# Autodesk Inventor assembly: Base Cover Assembly
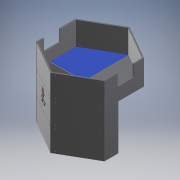
[picture p0: Inventor's stored thumbnail of the model, 180x180]
Saved by Autodesk Inventor 2017 (Build 210142000, 142)
## iProperties
Created: 2018-10-18
Part Number: Base Cover Assembly
Document SubType Name: Assembly
Designer: Dell
Author: Dell
## Documents named in this file (15)
- C:\Users\Dell\Documents\GitHub\tr2\Base\Base Cover Assembly.iam
- C:\Users\Dell\Documents\GitHub\tr2\Base\BA03.ipt
- C:\Users\Dell\Documents\GitHub\tr2\Base\BA04.ipt
- C:\Users\Dell\Documents\GitHub\tr2\Base\BA05.ipt
- C:\Users\Dell\Documents\GitHub\tr2\Base\BA09.ipt
- C:\Users\Dell\Documents\GitHub\tr2\Base\BA10.ipt
- C:\Users\Dell\Documents\GitHub\tr2\Base\BA12.ipt
- C:\Users\Dell\Documents\GitHub\tr2\Base\BA14.ipt
- C:\Users\Dell\Documents\GitHub\tr2\Base\Power Switch\Power Switch.iam
- C:\Users\Dell\Documents\GitHub\tr2\Base\Ethernet Port.ipt
- C:\Users\Dell\Documents\GitHub\tr2\Base\HDMI Port.ipt
- C:\Users\Dell\Documents\GitHub\tr2\Base\USB Hub.ipt
- C:\Users\Dell\Documents\GitHub\tr2\Base\BA19.ipt
- C:\Users\Dell\Documents\GitHub\tr2\Base\BA20.ipt
- C:\Users\Dell\Documents\GitHub\tr2\Base\BA21.ipt
## Components (24 placed, 14 different names)
1. BA03:1 — Mate:38, Mate:41, Flush:10, Mate:52, Mate:55
2. BA03:2 — Mate:20, Mate:43, Mate:44, Flush:10
3. BA03:3 — Mate:21, Mate:22, Mate:26, Mate:53
4. BA03:4 — Mate:17, Mate:19, Mate:21, Mate:23, Mate:64, Mate:65
5. BA04:1 — Mate:24, Mate:25, Mate:26, Mate:29, Mate:30
6. BA05:1 — Mate:18, Mate:19, Mate:20, Mate:23, Mate:27, Mate:66
7. BA03:5 — Mate:36, Mate:38, Mate:47
8. BA03:6 — Mate:41, Mate:49, Mate:81, Mate:83
9. BA03:7 — Mate:43, Mate:44, Mate:56, Mate:80
10. BA09:1 — Mate:29, Mate:30, Mate:33
11. BA09:4 — Mate:27, Mate:34, Mate:36
12. BA10:1 — Mate:17, Mate:18, Mate:22, Mate:24, Mate:25
13. BA10:2 — Mate:64, Mate:65, Mate:66
14. BA12:1 — Mate:33, Mate:54, Mate:75
15. BA12:2 — Mate:34, Mate:76
16. BA14:1 — Mate:47, Mate:49, Mate:55, Mate:56, Mate:57, Mate:58, Mate:59, Mate:67, Mate:68, Flush:11, Mate:69, Mate:70, Mate:71, Mate:72, Flush:12, Flush:13
17. Power Switch:1 [sub-assembly] — Mate:57, Mate:58, Mate:59
18. Ethernet Port:1 — Mate:69, Mate:72, Flush:13
19. HDMI Port:1 — Mate:70, Mate:71, Flush:12
20. USB Hub:1 — Mate:67, Mate:68, Flush:11
21. BA19:1 — Mate:75, Mate:78, Mate:85
22. BA19:2 — Mate:76, Mate:85
23. BA20:1 — Mate:78, Mate:80
24. BA21:1 — Mate:81, Mate:83
## Relationships (59: Mate 53, Flush 6)
- [Mate]: BA03:3 ↔ BA03:4
- [Mate]: BA03:2 ↔ BA03:5
- [Mate]: BA03:5 ↔ BA03:6
- [Mate]: BA04:1 ↔ BA09:1
- [Mate]: BA05:1 ↔ BA09:4
- [Mate]: BA04:1 ↔ BA12:1
- [Mate]: BA05:1 ↔ BA12:2
- [Flush]: BA09:4 ↔ BA12:2
- [Flush]: BA03:3 ↔ BA10:1
- Mate:17: BA03:4 ↔ BA10:1
- Mate:18: BA05:1 ↔ BA10:1
- Mate:19: BA03:4 ↔ BA05:1
- Mate:20: BA03:2 ↔ BA05:1
- Mate:21: BA03:3 ↔ BA03:4
- Mate:22: BA03:3 ↔ BA10:1
- Mate:23: BA03:4 ↔ BA05:1
- Mate:24: BA04:1 ↔ BA10:1
- Mate:25: BA04:1 ↔ BA10:1
- Mate:26: BA03:3 ↔ BA04:1
- Mate:27: BA05:1 ↔ BA09:4
- Mate:29: BA04:1 ↔ BA09:1
- Mate:30: BA04:1 ↔ BA09:1
- Mate:33: BA09:1 ↔ BA12:1
- Mate:34: BA09:4 ↔ BA12:2
- Mate:36: BA03:5 ↔ BA09:4
- Mate:38: BA03:1 ↔ BA03:5
- Mate:41: BA03:1 ↔ BA03:6
- Mate:43: BA03:2 ↔ BA03:7
- Mate:44: BA03:2 ↔ BA03:7
- Mate:47: BA03:5 ↔ BA14:1
- Mate:49: BA03:6 ↔ BA14:1
- Flush:10: BA03:1 ↔ BA03:2
- Mate:52: BA03:1
- Mate:53: BA03:3
- Mate:54: BA12:1
- Mate:55: BA03:1 ↔ BA14:1
- Mate:56: BA03:7 ↔ BA14:1
- Mate:57: BA14:1 ↔ Power Switch:1
- Mate:58: BA14:1 ↔ Power Switch:1
- Mate:59: BA14:1 ↔ Power Switch:1
- Mate:64: BA03:4 ↔ BA10:2
- Mate:65: BA03:4 ↔ BA10:2
- Mate:66: BA05:1 ↔ BA10:2
- Mate:67: BA14:1 ↔ USB Hub:1
- Mate:68: BA14:1 ↔ USB Hub:1
- Flush:11 (1 mm): BA14:1 ↔ USB Hub:1
- Mate:69: BA14:1 ↔ Ethernet Port:1
- Mate:70 (1 mm): BA14:1 ↔ HDMI Port:1
- Mate:71 (1 mm): BA14:1 ↔ HDMI Port:1
- Mate:72: BA14:1 ↔ Ethernet Port:1
- Flush:12: BA14:1 ↔ HDMI Port:1
- Flush:13: BA14:1 ↔ Ethernet Port:1
- Mate:75: BA12:1 ↔ BA19:1
- Mate:76: BA12:2 ↔ BA19:2
- Mate:78: BA19:1 ↔ BA20:1
- Mate:80: BA03:7 ↔ BA20:1
- Mate:81: BA03:6 ↔ BA21:1
- Mate:83: BA03:6 ↔ BA21:1
- Mate:85: BA19:1 ↔ BA19:2
